# Autodesk Inventor assembly: Assembly1
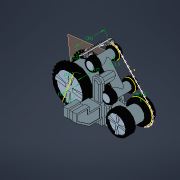
[picture p0: Inventor's stored thumbnail of the model, 180x180]
Saved by Autodesk Inventor 2022 (Build 260153000, 153)
## iProperties
Created: 2022-01-09
Part Number: Assembly1
Document SubType Name: Assembly
Designer: MatusBarany
Author: MatusBarany
## Documents named in this file (12)
- C:\Users\MatusBarany\Documents\Inventor\shortthinner\Assembly1.iam
- C:\Users\MatusBarany\Documents\Inventor\shortthinner\McCrea_chrbat_walle.ipt
- C:\Users\MatusBarany\Documents\Inventor\shortthinner\McCrea_diel_retaze_walle.ipt
- C:\Users\MatusBarany\Documents\Inventor\shortthinner\McCrea_male_koleso_walle.ipt
- C:\Users\MatusBarany\Documents\Inventor\shortthinner\McCrea_polspojka_stredne_koleso_walle.ipt
- C:\Users\MatusBarany\Documents\Inventor\shortthinner\McCrea_polspojka_velke_koleso_walle.ipt
- C:\Users\MatusBarany\Documents\Inventor\shortthinner\McCrea_spojka_male_koleso_walle.ipt
- C:\Users\MatusBarany\Documents\Inventor\shortthinner\McCrea_spojka_pasy_telo_walle.ipt
- C:\Users\MatusBarany\Documents\Inventor\shortthinner\McCrea_stredne_koleso_walle.ipt
- C:\Users\MatusBarany\Documents\Inventor\shortthinner\McCrea_uchytka_walle.ipt
- C:\Users\MatusBarany\Documents\Inventor\shortthinner\McCrea_velke_koleso_walle.ipt
- C:\Users\Public\Documents\Autodesk\Inventor 2022\McCrea_draha_walle.ipt
## Components (16 placed, 11 different names)
1. McCrea_chrbat_walle:3 — Mate:1, Rotational:1, Mate:2, Mate:3, Mate:4, Mate:5, Mate:6
2. McCrea_male_koleso_walle:1 — Rigid:4
3. McCrea_polspojka_stredne_koleso_walle:1 — Mate:8, Flush:1, Mate:9, Rigid:2, Rigid:3
4. McCrea_polspojka_velke_koleso_walle:1 — Rigid:1, Rotational:2, Cylindrical:1, Mate:7, Mate:8, Flush:1, Mate:9
5. McCrea_spojka_male_koleso_walle:1 — Rotational:1, Rigid:4, Rigid:5, Rigid:6, Rigid:7
6. McCrea_spojka_pasy_telo_walle:1 — Mate:1, Mate:5, Mate:6
7. McCrea_velke_koleso_walle:1 — Rigid:1
8. McCrea_velke_koleso_walle:2 — Rotational:2, Flush:2
9. McCrea_stredne_koleso_walle:2 — Rigid:3
10. McCrea_uchytka_walle:1 — Mate:2, Mate:3, Mate:4, Cylindrical:1, Mate:7
11. McCrea_male_koleso_walle:2 — Rigid:7
12. McCrea_stredne_koleso_walle:3 — Rigid:2
13. McCrea_male_koleso_walle:4 — Rigid:6
14. McCrea_male_koleso_walle:5 — Rigid:5
15. McCrea_draha_walle:1 — Flush:2, Mate:10, Mate:11, Mate:12
16. McCrea_diel_retaze_walle:1 — Mate:10, Mate:11, Mate:12
## Relationships (24: Mate 12, WeldJoint 7, RevoluteJoint 2, Flush 2, CylindricalJoint 1)
- Mate:1: McCrea_chrbat_walle:3 ↔ McCrea_spojka_pasy_telo_walle:1
- Rotational:1 [RevoluteJoint]: McCrea_chrbat_walle:3 ↔ McCrea_spojka_male_koleso_walle:1
- Rigid:1 [WeldJoint]: McCrea_polspojka_velke_koleso_walle:1 ↔ McCrea_velke_koleso_walle:1
- Rotational:2 [RevoluteJoint]: McCrea_polspojka_velke_koleso_walle:1 ↔ McCrea_velke_koleso_walle:2
- Mate:2: McCrea_chrbat_walle:3 ↔ McCrea_uchytka_walle:1
- Mate:3: McCrea_chrbat_walle:3 ↔ McCrea_uchytka_walle:1
- Mate:4: McCrea_chrbat_walle:3 ↔ McCrea_uchytka_walle:1
- Mate:5: McCrea_chrbat_walle:3 ↔ McCrea_spojka_pasy_telo_walle:1
- Mate:6: McCrea_chrbat_walle:3 ↔ McCrea_spojka_pasy_telo_walle:1
- Cylindrical:1: McCrea_polspojka_velke_koleso_walle:1 ↔ McCrea_uchytka_walle:1
- Mate:7: McCrea_polspojka_velke_koleso_walle:1 ↔ McCrea_uchytka_walle:1
- Mate:8: McCrea_polspojka_stredne_koleso_walle:1 ↔ McCrea_polspojka_velke_koleso_walle:1
- Flush:1: McCrea_polspojka_stredne_koleso_walle:1 ↔ McCrea_polspojka_velke_koleso_walle:1
- Mate:9: McCrea_polspojka_stredne_koleso_walle:1 ↔ McCrea_polspojka_velke_koleso_walle:1
- Rigid:2 [WeldJoint]: McCrea_polspojka_stredne_koleso_walle:1 ↔ McCrea_stredne_koleso_walle:3
- Rigid:3 [WeldJoint]: McCrea_polspojka_stredne_koleso_walle:1 ↔ McCrea_stredne_koleso_walle:2
- Rigid:4 [WeldJoint]: McCrea_male_koleso_walle:1 ↔ McCrea_spojka_male_koleso_walle:1
- Rigid:5 [WeldJoint]: McCrea_spojka_male_koleso_walle:1 ↔ McCrea_male_koleso_walle:5
- Rigid:6 [WeldJoint]: McCrea_spojka_male_koleso_walle:1 ↔ McCrea_male_koleso_walle:4
- Rigid:7 [WeldJoint]: McCrea_spojka_male_koleso_walle:1 ↔ McCrea_male_koleso_walle:2
- Flush:2 (-1.4986 mm): McCrea_velke_koleso_walle:2 ↔ McCrea_draha_walle:1
- Mate:10: McCrea_draha_walle:1 ↔ McCrea_diel_retaze_walle:1
- Mate:11: McCrea_draha_walle:1 ↔ McCrea_diel_retaze_walle:1
- Mate:12: McCrea_draha_walle:1 ↔ McCrea_diel_retaze_walle:1
